# Autodesk Inventor assembly: BangTai_Lap
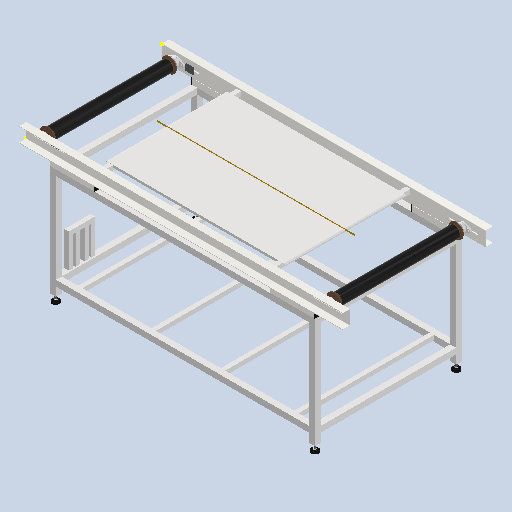
[picture p0: Inventor's stored thumbnail of the model, 512x512]
Saved by Autodesk Inventor 2023 (Build 270158000, 158)
## iProperties
Created: 2025-04-17
Part Number: BangTai_Lap
Document SubType Name: Assembly
Designer: huyqu
Author: huyqu
## Documents named in this file (9)
- E:\TAI LIEU\Final_Project\DONE\Bangtai\BangTai_Lap.iam
- E:\TAI LIEU\Final_Project\DONE\Bangtai\BangTai.ipt
- E:\TAI LIEU\Final_Project\DONE\Bangtai\InoxLienKet.ipt
- E:\TAI LIEU\Final_Project\DONE\Bangtai\ThanhKe.ipt
- E:\TAI LIEU\Final_Project\DONE\Bangtai\Nhom30.ipt
- E:\TAI LIEU\Final_Project\DONE\Bangtai\CoDinhDiChuyenBT.ipt
- E:\TAI LIEU\Final_Project\DONE\Bangtai\ChanBangTai.ipt
- E:\TAI LIEU\Final_Project\DONE\Bangtai\Ke_Bang_Tai.ipt
- E:\TAI LIEU\Final_Project\DONE\BangTai\Rolo_Lap.iam
## Components (17 placed, 8 different names)
1. BangTai:1 — Mate:1, Flush:1, Flush:2, Mate:2, Flush:3, Flush:4, Mate:3, Flush:5, Flush:6, Mate:4, Flush:7, Flush:8, Flush:10, Flush:12, Mate:15, Angle:1, Mate:16, Mate:17, Mate:18
2. InoxLienKet:1 — Mate:2, Flush:3, Flush:4, Mate:6, Flush:11
3. InoxLienKet:2 — Mate:1, Flush:1, Flush:2
4. InoxLienKet:3 — Mate:4, Flush:7, Flush:8, Mate:5, Flush:9
5. InoxLienKet:4 — Mate:3, Flush:5, Flush:6
6. ThanhKe:1 — Mate:6, Flush:11, Flush:12, Mate:13, Flush:19, Flush:20, Mate:35, Mate:36
7. ThanhKe:2 — Mate:5, Flush:9, Flush:10, Mate:7, Flush:13, Flush:18, Mate:14, Flush:21, Flush:22, Mate:20, Mate:34, Flush:25, Flush:26
8. Nhom30:3 — Mate:7, Flush:13, Flush:18, Mate:19, Mate:21
9. CoDinhDiChuyenBT:1 — Mate:13, Flush:19, Flush:20
10. CoDinhDiChuyenBT:2 — Mate:14, Flush:21, Flush:22
11. ChanBangTai:1 — Mate:18
12. ChanBangTai:2 — Mate:17
13. ChanBangTai:3 — Mate:16
14. ChanBangTai:4 — Mate:15, Angle:1
15. Ke_Bang_Tai:1 — Mate:19, Mate:20, Mate:21
16. Nhom30:4 — Mate:34, Flush:25, Flush:26
17. Rolo_Lap:1 [sub-assembly] — Mate:35, Mate:36
## Relationships (40: Flush 20, Mate 19, Angle 1)
- Mate:1: BangTai:1 ↔ InoxLienKet:2
- Flush:1: BangTai:1 ↔ InoxLienKet:2
- Flush:2: BangTai:1 ↔ InoxLienKet:2
- Mate:2: BangTai:1 ↔ InoxLienKet:1
- Flush:3: BangTai:1 ↔ InoxLienKet:1
- Flush:4: BangTai:1 ↔ InoxLienKet:1
- Mate:3: BangTai:1 ↔ InoxLienKet:4
- Flush:5: BangTai:1 ↔ InoxLienKet:4
- Flush:6: BangTai:1 ↔ InoxLienKet:4
- Mate:4: BangTai:1 ↔ InoxLienKet:3
- Flush:7: BangTai:1 ↔ InoxLienKet:3
- Flush:8: BangTai:1 ↔ InoxLienKet:3
- Mate:5: InoxLienKet:3 ↔ ThanhKe:2
- Flush:9: InoxLienKet:3 ↔ ThanhKe:2
- Flush:10 (-200 mm): BangTai:1 ↔ ThanhKe:2
- Mate:6: InoxLienKet:1 ↔ ThanhKe:1
- Flush:11: InoxLienKet:1 ↔ ThanhKe:1
- Flush:12 (-200 mm): BangTai:1 ↔ ThanhKe:1
- Mate:7: ThanhKe:2 ↔ Nhom30:3
- Flush:13 (10 mm): ThanhKe:2 ↔ Nhom30:3
- Flush:18 (510 mm): ThanhKe:2 ↔ Nhom30:3
- Mate:13: ThanhKe:1 ↔ CoDinhDiChuyenBT:1
- Flush:19 (30 mm): ThanhKe:1 ↔ CoDinhDiChuyenBT:1
- Flush:20 (170 mm): ThanhKe:1 ↔ CoDinhDiChuyenBT:1
- Mate:14: ThanhKe:2 ↔ CoDinhDiChuyenBT:2
- Flush:21 (-30 mm): ThanhKe:2 ↔ CoDinhDiChuyenBT:2
- Flush:22 (170 mm): ThanhKe:2 ↔ CoDinhDiChuyenBT:2
- Mate:15: BangTai:1 ↔ ChanBangTai:4
- Angle:1 (0 deg): BangTai:1 ↔ ChanBangTai:4
- Mate:16: BangTai:1 ↔ ChanBangTai:3
- Mate:17: BangTai:1 ↔ ChanBangTai:2
- Mate:18: BangTai:1 ↔ ChanBangTai:1
- Mate:19: Nhom30:3 ↔ Ke_Bang_Tai:1
- Mate:20 (50 mm): ThanhKe:2 ↔ Ke_Bang_Tai:1
- Mate:21 (10 mm): Nhom30:3 ↔ Ke_Bang_Tai:1
- Mate:34: ThanhKe:2 ↔ Nhom30:4
- Flush:25 (10 mm): ThanhKe:2 ↔ Nhom30:4
- Flush:26 (510 mm): ThanhKe:2 ↔ Nhom30:4
- Mate:35: ThanhKe:1 ↔ Rolo_Lap:1
- Mate:36: ThanhKe:1 ↔ Rolo_Lap:1
